# Autodesk Inventor assembly: Chuck with Glue Reservoir Plate
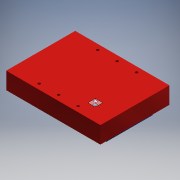
[picture p0: Inventor's stored thumbnail of the model, 180x180]
Saved by Autodesk Inventor 2019.4 (Build 234330000, 330)
## iProperties
Created: 2021-01-11
Part Number: Chuck with Glue Reservoir Plate
Document SubType Name: Assembly
Designer: caleb
Author: caleb
## Documents named in this file (3)
- C:\Users\cfang\Desktop\nebraska-silicon-lab\CAD\ETL\Module Assembly\Chuck with Glue Reservoir Plate.iam
- C:\Users\cfang\Desktop\nebraska-silicon-lab\CAD\ETL\Module Assembly\Chuck\Chuck Assembly.iam
- C:\Users\cfang\Desktop\nebraska-silicon-lab\CAD\ETL\Module Assembly\Glue Reservoir Plate\Glue Reservoir Plate.ipt
## Components (2 placed, 2 different names)
1. Chuck Assembly:1 [sub-assembly] — Mate:1, Tangent:1, Tangent:2, Tangent:3
2. Glue Reservoir Plate:1 — Mate:1, Tangent:1, Tangent:2, Tangent:3
## Relationships (4: Tangent 3, Mate 1)
- Mate:1: Chuck Assembly:1 ↔ Glue Reservoir Plate:1
- Tangent:1: Chuck Assembly:1 ↔ Glue Reservoir Plate:1
- Tangent:2: Chuck Assembly:1 ↔ Glue Reservoir Plate:1
- Tangent:3: Chuck Assembly:1 ↔ Glue Reservoir Plate:1
